# Autodesk Inventor assembly: Z-AXIS ASSEMBLY V2.1
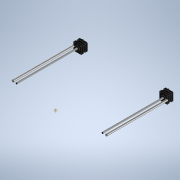
[picture p0: Inventor's stored thumbnail of the model, 180x180]
Saved by Autodesk Inventor 2020.3 (Build 243373010, 373A)
## iProperties
Created: 2019-09-17
Part Number: Z-AXIS ASSEMBLY V2.1
Document SubType Name: Assembly
Designer: pepd9
Author: pepd9
## Documents named in this file (4)
- D:\Designs\MK3PRO P1\Z-Axis\Z-AXIS ASSEMBLY V2.1.iam
- D:\Designs\MK3PRO P1\Z-Axis\Z-axis_motor_L.ipt
- D:\Designs\MK3PRO P1\Z-Axis\Z-axis_motor_R.ipt
- D:\Designs\MK3PRO P1\Z-Axis\Z-Axis Rod.ipt
## Components (4 placed, 3 different names)
1. Z-Axis Rod:1 — Mate:11, Mate:16
2. Z-Axis Rod:2 — Mate:12, Mate:17
3. Z-axis_motor_L:1 — Mate:6, Angle:1, Flush:3, Flush:4, Mate:15, Mate:16
4. Z-axis_motor_R:1 — Mate:5, Flush:3, Flush:4, Mate:17
## Relationships (22: Mate 15, Flush 6, Angle 1)
- Flush:1 (225 mm)
- Flush:2 (-225 mm)
- Mate:1
- Mate:2
- Mate:3
- Mate:4
- Mate:5: Z-axis_motor_R:1
- Mate:6: Z-axis_motor_L:1
- Angle:1 (180 deg): Z-axis_motor_L:1
- Flush:3: Z-axis_motor_L:1 ↔ Z-axis_motor_R:1
- Flush:4: Z-axis_motor_L:1 ↔ Z-axis_motor_R:1
- Flush:5 (-20 mm)
- Flush:6 (20 mm)
- Mate:7
- Mate:8
- Mate:9
- Mate:10
- Mate:11: Z-Axis Rod:1
- Mate:12: Z-Axis Rod:2
- Mate:15 (340 mm): Z-axis_motor_L:1
- Mate:16: Z-Axis Rod:1 ↔ Z-axis_motor_L:1
- Mate:17: Z-Axis Rod:2 ↔ Z-axis_motor_R:1
